# Autodesk Inventor assembly: Drone Assembly
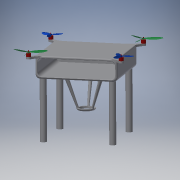
[picture p0: Inventor's stored thumbnail of the model, 180x180]
Saved by Autodesk Inventor 2019 (Build 230136000, 136)
## iProperties
Created: 2020-03-20
Part Number: Drone Assembly
Document SubType Name: Assembly
Designer: 18186
Author: 18186
## Documents named in this file (7)
- D:\Food Delivery Drone\Drone Assembly.iam
- D:\Food Delivery Drone\Drone Body.ipt
- D:\Food Delivery Drone\motor mock.ipt
- D:\Food Delivery Drone\PropellerCCW-3Blade.ipt
- D:\Food Delivery Drone\PropellerCW-3Blade.ipt
- D:\Food Delivery Drone\Drone Body Cupholder.ipt
- D:\Food Delivery Drone\Drone Body Leg.ipt
## Components (14 placed, 6 different names)
1. Drone Body:1 — Mate:17, Mate:18, Mate:19, Mate:20, Mate:21, Mate:22, Mate:23, Mate:24, Mate:29, Tangent:1, Mate:30, Mate:31, Mate:32, Mate:33, Mate:34, Mate:35, Mate:36, Mate:37, Mate:38
2. motor mock:1 — Mate:21, Mate:22, Mate:27, Mate:28
3. motor mock:2 — Mate:17, Mate:18, Mate:25, Mate:26
4. motor mock:3 — Mate:11, Mate:12, Mate:19, Mate:20
5. motor mock:4 — Mate:9, Mate:10, Mate:23, Mate:24
6. PropellerCCW-3Blade:1 — Mate:11, Mate:12
7. PropellerCCW-3Blade:2 — Mate:9, Mate:10
8. PropellerCW-3Blade:1 — Mate:27, Mate:28
9. PropellerCW-3Blade:2 — Mate:25, Mate:26
10. Drone Body Cupholder:1 — Mate:29, Tangent:1, Mate:30
11. Drone Body Leg:1 — Mate:37, Mate:38
12. Drone Body Leg:2 — Mate:35, Mate:36
13. Drone Body Leg:3 — Mate:31, Mate:32
14. Drone Body Leg:4 — Mate:33, Mate:34
## Relationships (27: Mate 26, Tangent 1)
- Mate:9: motor mock:4 ↔ PropellerCCW-3Blade:2
- Mate:10: motor mock:4 ↔ PropellerCCW-3Blade:2
- Mate:11: motor mock:3 ↔ PropellerCCW-3Blade:1
- Mate:12: motor mock:3 ↔ PropellerCCW-3Blade:1
- Mate:17: Drone Body:1 ↔ motor mock:2
- Mate:18: Drone Body:1 ↔ motor mock:2
- Mate:19: Drone Body:1 ↔ motor mock:3
- Mate:20: Drone Body:1 ↔ motor mock:3
- Mate:21: Drone Body:1 ↔ motor mock:1
- Mate:22: Drone Body:1 ↔ motor mock:1
- Mate:23: Drone Body:1 ↔ motor mock:4
- Mate:24: Drone Body:1 ↔ motor mock:4
- Mate:25: motor mock:2 ↔ PropellerCW-3Blade:2
- Mate:26: motor mock:2 ↔ PropellerCW-3Blade:2
- Mate:27: motor mock:1 ↔ PropellerCW-3Blade:1
- Mate:28: motor mock:1 ↔ PropellerCW-3Blade:1
- Mate:29: Drone Body:1 ↔ Drone Body Cupholder:1
- Tangent:1: Drone Body:1 ↔ Drone Body Cupholder:1
- Mate:30: Drone Body:1 ↔ Drone Body Cupholder:1
- Mate:31: Drone Body:1 ↔ Drone Body Leg:3
- Mate:32: Drone Body:1 ↔ Drone Body Leg:3
- Mate:33: Drone Body:1 ↔ Drone Body Leg:4
- Mate:34: Drone Body:1 ↔ Drone Body Leg:4
- Mate:35: Drone Body:1 ↔ Drone Body Leg:2
- Mate:36: Drone Body:1 ↔ Drone Body Leg:2
- Mate:37: Drone Body:1 ↔ Drone Body Leg:1
- Mate:38: Drone Body:1 ↔ Drone Body Leg:1
